# Autodesk Inventor assembly: mainflap_center
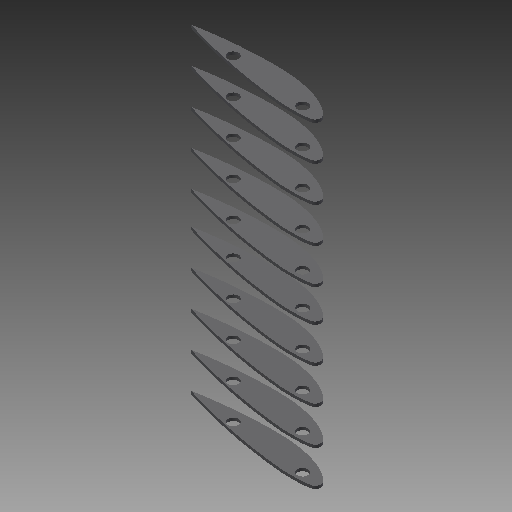
[picture p0: Inventor's stored thumbnail of the model, 512x512]
Saved by Autodesk Inventor 2018.2 (Build 222227000, 227)
## iProperties
Created: 2018-03-05
Part Number: mainflap_center
Material: 一般
Document SubType Name: Assembly
Designer: ku_sk
Author: ku_sk
## Documents named in this file (2)
- C:\Users\ku_sk\Documents\Inventor\Aero\KS-15\Fr.wing\parts\mainflap_center\mainflap_center.iam
- C:\Users\ku_sk\Documents\Inventor\Aero\KS-15\Fr.wing\parts\mainflap_center\plate_mc.ipt
## Components (10 placed, 1 different names)
1. plate_mc:1 — フラッシュ:1, メイト:3, メイト:4
2. plate_mc:2 — メイト:1, メイト:2, メイト:3, メイト:4, フラッシュ:2, メイト:5, メイト:6
3. plate_mc:3 — フラッシュ:2, フラッシュ:3, メイト:5, メイト:6, メイト:7, メイト:8
4. plate_mc:4 — フラッシュ:3, フラッシュ:4, メイト:7, メイト:8, メイト:9, メイト:10
5. plate_mc:5 — フラッシュ:4, フラッシュ:5, メイト:9, メイト:10, メイト:11, メイト:12
6. plate_mc:6 — フラッシュ:5, フラッシュ:6, メイト:11, メイト:12, メイト:13, メイト:14
7. plate_mc:7 — フラッシュ:6, フラッシュ:7, メイト:13, メイト:14, メイト:15, メイト:16
8. plate_mc:8 — フラッシュ:7, メイト:15, メイト:16, フラッシュ:8, メイト:17, メイト:18
9. plate_mc:9 — フラッシュ:8, フラッシュ:9, メイト:17, メイト:18, メイト:19
10. plate_mc:10 — フラッシュ:9, メイト:19
## Relationships (28: Mate 19, Flush 9)
- フラッシュ:1 [Flush] (-225 mm): plate_mc:1
- メイト:1 [Mate] (-225 mm): plate_mc:2
- メイト:2 [Mate]: plate_mc:2
- メイト:3 [Mate]: plate_mc:1 ↔ plate_mc:2
- メイト:4 [Mate]: plate_mc:1 ↔ plate_mc:2
- フラッシュ:2 [Flush] (50 mm): plate_mc:2 ↔ plate_mc:3
- フラッシュ:3 [Flush] (-50 mm): plate_mc:3 ↔ plate_mc:4
- フラッシュ:4 [Flush] (50 mm): plate_mc:4 ↔ plate_mc:5
- フラッシュ:5 [Flush] (-50 mm): plate_mc:5 ↔ plate_mc:6
- フラッシュ:6 [Flush] (-46 mm): plate_mc:6 ↔ plate_mc:7
- フラッシュ:7 [Flush] (-50 mm): plate_mc:7 ↔ plate_mc:8
- メイト:5 [Mate]: plate_mc:2 ↔ plate_mc:3
- メイト:6 [Mate]: plate_mc:2 ↔ plate_mc:3
- メイト:7 [Mate]: plate_mc:3 ↔ plate_mc:4
- メイト:8 [Mate]: plate_mc:3 ↔ plate_mc:4
- メイト:9 [Mate]: plate_mc:4 ↔ plate_mc:5
- メイト:10 [Mate]: plate_mc:4 ↔ plate_mc:5
- メイト:11 [Mate]: plate_mc:5 ↔ plate_mc:6
- メイト:12 [Mate]: plate_mc:5 ↔ plate_mc:6
- メイト:13 [Mate]: plate_mc:6 ↔ plate_mc:7
- メイト:14 [Mate]: plate_mc:6 ↔ plate_mc:7
- メイト:15 [Mate]: plate_mc:7 ↔ plate_mc:8
- メイト:16 [Mate]: plate_mc:7 ↔ plate_mc:8
- フラッシュ:8 [Flush] (-50 mm): plate_mc:8 ↔ plate_mc:9
- フラッシュ:9 [Flush] (-50 mm): plate_mc:9 ↔ plate_mc:10
- メイト:17 [Mate]: plate_mc:8 ↔ plate_mc:9
- メイト:18 [Mate]: plate_mc:8 ↔ plate_mc:9
- メイト:19 [Mate]: plate_mc:9 ↔ plate_mc:10
